# Autodesk Inventor assembly: RoboTTInventorAssambly
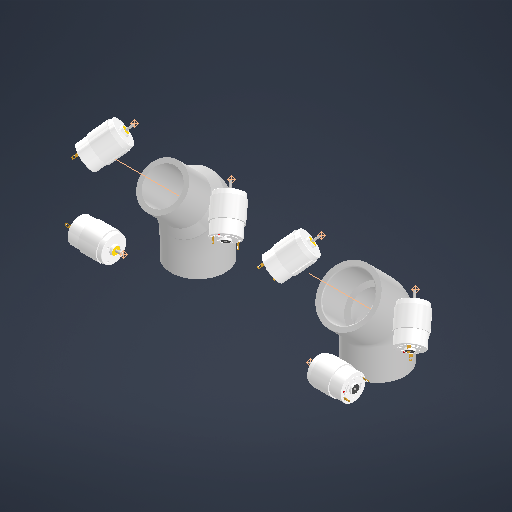
[picture p0: Inventor's stored thumbnail of the model, 512x512]
Saved by Autodesk Inventor 2026 (Build 300175050, 175E)
## iProperties
Created: 2025-06-23
Part Number: RoboTTInventorAssambly
Document SubType Name: Assembly
Designer: RubenPC
Author: RubenPC
## Documents named in this file (4)
- C:\Users\RubenPC\Code\RoboTT\assets\RoboTTInventorAssambly.iam
- C:\Users\RubenPC\Code\RoboTT\assets\MABUCHI_MOTOR_385\MABUCHI_MOTOR_385\MABUCHI_MOTOR_385.ipt
- C:\Users\RubenPC\Code\RoboTT\assets\CurvePVC45\CurvePVC45\CurvePVC45.ipt
- C:\Users\RubenPC\Code\RoboTT\assets\CurvePVC45MaleFamale\CurvePVC45MaleFamale\CurvePVC45MaleFamale.ipt
## Components (8 placed, 3 different names)
1. MABUCHI_MOTOR_385:1 — Mate:16, Mate:25, Flush:4
2. MABUCHI_MOTOR_385:2 — Mate:14, Mate:24, Flush:5
3. MABUCHI_MOTOR_385:3 — Mate:15, Mate:23, Flush:6
4. CurvePVC45:1 — Mate:6, Mate:9, Mate:11, Flush:3, Mate:13, Mate:14, Mate:15, Mate:16, Mate:17, Mate:18, Mate:19, Mate:20, Mate:21, Mate:22, Mate:23, Mate:24, Mate:25
5. CurvePVC45MaleFamale:1 — Mate:3, Mate:7, Mate:10, Flush:3, Mate:13
6. MABUCHI_MOTOR_385:4 — Mate:19, Mate:22
7. MABUCHI_MOTOR_385:5 — Mate:18, Mate:21
8. MABUCHI_MOTOR_385:6 — Mate:17, Mate:20
## Relationships (23: Mate 19, Flush 4)
- Mate:3: CurvePVC45MaleFamale:1
- Mate:6: CurvePVC45:1
- Mate:7: CurvePVC45MaleFamale:1
- Mate:9 (200 mm): CurvePVC45:1
- Mate:10: CurvePVC45MaleFamale:1
- Mate:11: CurvePVC45:1
- Flush:3: CurvePVC45:1 ↔ CurvePVC45MaleFamale:1
- Mate:13: CurvePVC45:1 ↔ CurvePVC45MaleFamale:1
- Mate:14: MABUCHI_MOTOR_385:2 ↔ CurvePVC45:1
- Mate:15: MABUCHI_MOTOR_385:3 ↔ CurvePVC45:1
- Mate:16: MABUCHI_MOTOR_385:1 ↔ CurvePVC45:1
- Mate:17: CurvePVC45:1 ↔ MABUCHI_MOTOR_385:6
- Mate:18: CurvePVC45:1 ↔ MABUCHI_MOTOR_385:5
- Mate:19: CurvePVC45:1 ↔ MABUCHI_MOTOR_385:4
- Mate:20: CurvePVC45:1 ↔ MABUCHI_MOTOR_385:6
- Mate:21: CurvePVC45:1 ↔ MABUCHI_MOTOR_385:5
- Mate:22: CurvePVC45:1 ↔ MABUCHI_MOTOR_385:4
- Mate:23: MABUCHI_MOTOR_385:3 ↔ CurvePVC45:1
- Mate:24: MABUCHI_MOTOR_385:2 ↔ CurvePVC45:1
- Mate:25: MABUCHI_MOTOR_385:1 ↔ CurvePVC45:1
- Flush:4: MABUCHI_MOTOR_385:1
- Flush:5: MABUCHI_MOTOR_385:2
- Flush:6: MABUCHI_MOTOR_385:3
